# Autodesk Inventor assembly: 305-01
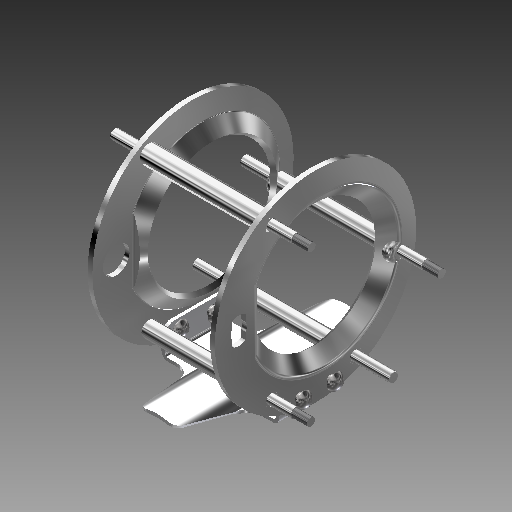
[picture p0: Inventor's stored thumbnail of the model, 512x512]
Saved by Autodesk Inventor 2019 (Build 230136000, 136)
## iProperties
Company: Autodesk Inc.
Created: 2012-01-24
Part Number: 305-01
Document SubType Name: Assembly
Designer: Autodesk Inc.
Mass: 33.0407 g
Surface Area: 171.485 cm^2
Volume: 11.6968 cm^3
Density: 2.82478 g/cm^3
Author: Inventor
## Documents named in this file (8)
- C:\TEMP\Fishing Rod\Workspaces\Reel Cage Assembly.iam
- C:\TEMP\Fishing Rod\Workspaces\Slotted Strut.ipt
- C:\TEMP\Fishing Rod\Workspaces\Spool Frame Ring - Back.ipt
- C:\TEMP\Fishing Rod\Workspaces\Spool Frame Ring - Front.ipt
- C:\TEMP\Fishing Rod\Workspaces\Strut.ipt
- C:\TEMP\Fishing Rod\Workspaces\Threaded Strut.ipt
- C:\TEMP\Fishing Rod\Workspaces\Mounting Bracket.ipt
- C:\TEMP\Fishing Rod\Workspaces\CNS 7339 - 3 x 8 x 2.5.ipt
## Components (11 placed, 7 different names)
1. Slotted Strut:1 — Insert:1, Angle:2, Flush:7
2. Spool Frame Ring - Back:1 — Insert:1, Insert:2, Insert:3, Insert:4, Mate:1, Angle:2, Mate:3, Mate:4, Mate:5, Insert:11
3. Spool Frame Ring - Front:1 — Mate:13, Mate:6, Flush:7
4. Strut:1 — Insert:4, Mate:6
5. Threaded Strut:1 — Insert:2, Mate:13
6. Threaded Strut:2 — Insert:3
7. Mounting Bracket:1 — Mate:3, Mate:4, Flush:6, Insert:8, Mate:5, Insert:9, Insert:10
8. CNS 7339 - 3 x 8 x 2.5:1 — Insert:8
9. CNS 7339 - 3 x 8 x 2.5:1 — Insert:9
10. CNS 7339 - 3 x 8 x 2.5:2 — Insert:10
11. CNS 7339 - 3 x 8 x 2.5:2 — Insert:11
## Relationships (17: Insert 8, Mate 6, Flush 2, Angle 1)
- Insert:1: Slotted Strut:1 ↔ Spool Frame Ring - Back:1
- Insert:2: Spool Frame Ring - Back:1 ↔ Threaded Strut:1
- Insert:3: Spool Frame Ring - Back:1 ↔ Threaded Strut:2
- Insert:4: Spool Frame Ring - Back:1 ↔ Strut:1
- Mate:1: Spool Frame Ring - Back:1
- Angle:2 (0 deg): Slotted Strut:1 ↔ Spool Frame Ring - Back:1
- Mate:3: Spool Frame Ring - Back:1 ↔ Mounting Bracket:1
- Mate:4: Spool Frame Ring - Back:1 ↔ Mounting Bracket:1
- Flush:6: Mounting Bracket:1
- Insert:8: Mounting Bracket:1 ↔ CNS 7339 - 3 x 8 x 2.5:1
- Insert:9: Mounting Bracket:1 ↔ CNS 7339 - 3 x 8 x 2.5:1
- Insert:10: Mounting Bracket:1 ↔ CNS 7339 - 3 x 8 x 2.5:2
- Mate:5: Spool Frame Ring - Back:1 ↔ Mounting Bracket:1
- Insert:11: Spool Frame Ring - Back:1 ↔ CNS 7339 - 3 x 8 x 2.5:2
- Mate:13: Spool Frame Ring - Front:1 ↔ Threaded Strut:1
- Mate:6: Spool Frame Ring - Front:1 ↔ Strut:1
- Flush:7: Slotted Strut:1 ↔ Spool Frame Ring - Front:1
